# Autodesk Inventor assembly: Torre Pont+Motor
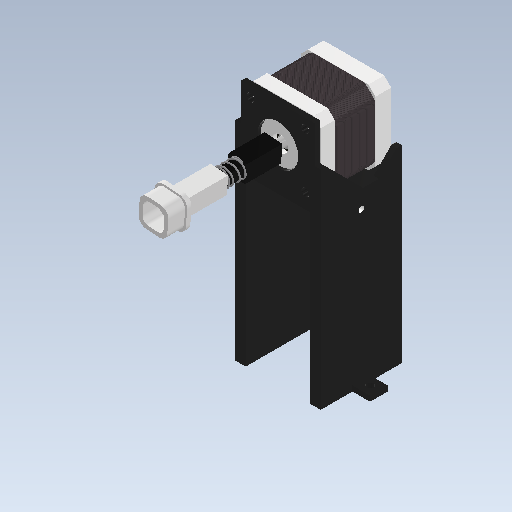
[picture p0: Inventor's stored thumbnail of the model, 512x512]
Saved by Autodesk Inventor 2021 (Build 250183000, 183)
## iProperties
Created: 2021-04-15
Part Number: Torre Pont+Motor
Document SubType Name: Assembly
Designer: Marc
Author: Marc
## Documents named in this file (6)
- C:\Users\Marc\Documents\Projectes\Rubik's Cube Solver\Prototip Definitiu\Torre Pont+Motor.iam
- C:\Users\Marc\Documents\Projectes\Rubik's Cube Solver\Prototip Definitiu\Components\Torre Motor Definitiva Pont.ipt
- C:\Users\Marc\Documents\Projectes\Rubik's Cube Solver\Prototip Definitiu\Components\Nema17\Steppermotor 17HS4417 1.7A 1.8° 2.55V v6_TOP.iam
- C:\Users\Marc\Documents\Projectes\Rubik's Cube Solver\Prototip Definitiu\Components\eixmobiblequadrat.ipt
- C:\Users\Marc\Documents\Projectes\Rubik's Cube Solver\Prototip Definitiu\Components\Molla Sodemann C04200350880S.ipt
- C:\Users\Marc\Documents\Projectes\Rubik's Cube Solver\Prototip Definitiu\Components\Eix Torres.ipt
## Components (5 placed, 5 different names)
1. Torre Motor Definitiva Pont:1 — Coincidencia:1, Coincidencia:2, Coincidencia:3
2. Steppermotor 17HS4417 1.7A 1.8° 2.55V v6_TOP:1 [sub-assembly] — Coincidencia:1, Coincidencia:2, Coincidencia:3, Coincidencia:4, Coincidencia:5
3. eixmobiblequadrat:1 — Coincidencia:4, Coincidencia:5, Coincidencia:6, Coincidencia:8
4. Molla Sodemann C04200350880S:1 — Coincidencia:6, Coincidencia:7
5. Eix Torres:1 — Coincidencia:7, Coincidencia:8
## Relationships (8: Mate 8)
- Coincidencia:1 [Mate]: Torre Motor Definitiva Pont:1 ↔ Steppermotor 17HS4417 1.7A 1.8° 2.55V v6_TOP:1
- Coincidencia:2 [Mate]: Torre Motor Definitiva Pont:1 ↔ Steppermotor 17HS4417 1.7A 1.8° 2.55V v6_TOP:1
- Coincidencia:3 [Mate] (0.25 mm): Torre Motor Definitiva Pont:1 ↔ Steppermotor 17HS4417 1.7A 1.8° 2.55V v6_TOP:1
- Coincidencia:4 [Mate]: Steppermotor 17HS4417 1.7A 1.8° 2.55V v6_TOP:1 ↔ eixmobiblequadrat:1
- Coincidencia:5 [Mate]: Steppermotor 17HS4417 1.7A 1.8° 2.55V v6_TOP:1 ↔ eixmobiblequadrat:1
- Coincidencia:6 [Mate]: eixmobiblequadrat:1 ↔ Molla Sodemann C04200350880S:1
- Coincidencia:7 [Mate]: Molla Sodemann C04200350880S:1 ↔ Eix Torres:1
- Coincidencia:8 [Mate]: eixmobiblequadrat:1 ↔ Eix Torres:1
